# Autodesk Inventor assembly: sensor_package6solar
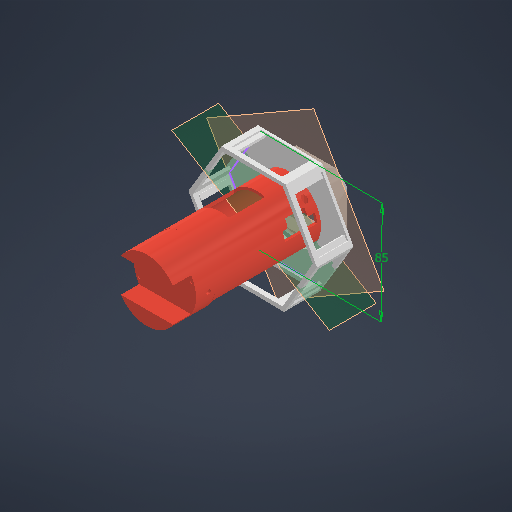
[picture p0: Inventor's stored thumbnail of the model, 512x512]
Saved by Autodesk Inventor 2027 (Build 310192060, 192F)
## iProperties
Created: 2026-07-17
Part Number: sensor_package6solar
Document SubType Name: Assembly
Designer: farde
Author: farde
## Documents named in this file (4)
- C:\Users\farde\Downloads\sensor_package6solar.iam
- C:\Users\farde\Downloads\sensor frame (1)\Part4.ipt
- C:\Users\farde\Downloads\sensor frame (1)\Part1.ipt
- C:\Users\farde\Downloads\part_lower.ipt
## Components (3 placed, 3 different names)
1. Part4:1 — Rigid:1, Rigid:2
2. part_lower:1 — Rigid:1
3. Part1:1 — Rigid:2
## Relationships (2: WeldJoint 2)
- Rigid:1 [WeldJoint] (-1.27 mm): Part4:1 ↔ part_lower:1
- Rigid:2 [WeldJoint] (1.27 mm): Part4:1 ↔ Part1:1
